# Autodesk Inventor assembly: finalassy
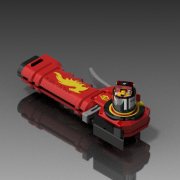
[picture p0: Inventor's stored thumbnail of the model, 180x180]
Saved by Autodesk Inventor 2018 (Build 220112000, 112)
## iProperties
Created: 2019-02-22
Part Number: finalassy
Material: 一般
Document SubType Name: Assembly
Designer: ku_sk
Author: ku_sk
## Documents named in this file (21)
- E:\windows\Documents\Inventor\Content Center Files\bay shooter\parts\finalassy.iam
- E:\windows\Documents\Inventor\Content Center Files\bay shooter\parts\undercover_modified.ipt
- E:\windows\Documents\Inventor\Content Center Files\bay shooter\parts\battery.ipt
- E:\windows\Documents\Inventor\Content Center Files\bay shooter\parts\brake.ipt
- E:\windows\Documents\Inventor\Content Center Files\bay shooter\parts\bay conect.ipt
- E:\windows\Documents\Inventor\Content Center Files\bay shooter\parts\bearing.ipt
- E:\windows\Documents\Inventor\Content Center Files\bay shooter\parts\bar.ipt
- E:\windows\Documents\Inventor\Content Center Files\bay shooter\parts\topcover.ipt
- E:\windows\Documents\Inventor\Content Center Files\bay shooter\parts\bar2.ipt
- E:\windows\Documents\Inventor\Content Center Files\bay shooter\parts\joint.ipt
- E:\windows\Documents\Inventor\Content Center Files\bay shooter\parts\switch.ipt
- E:\windows\Documents\Inventor\Content Center Files\bay shooter\parts\cover.ipt
- E:\windows\Documents\Inventor\Content Center Files\bay shooter\parts\ring.ipt
- E:\windows\Documents\Inventor\Content Center Files\bay shooter\parts\circuitcover.ipt
- E:\windows\Documents\Inventor\Content Center Files\bay shooter\parts\circuitcover1.ipt
- E:\windows\Documents\Inventor\Content Center Files\bay shooter\parts\gear.ipt
- E:\windows\Documents\Inventor\Content Center Files\bay shooter\parts\dragon.ipt
- E:\windows\Documents\Inventor\Content Center Files\bay shooter\parts\dragon_MIR.ipt
- E:\windows\Documents\Inventor\Content Center Files\bay shooter\parts\skyrimlogo2_1_9.ipt
- E:\windows\Documents\Inventor\Content Center Files\bay shooter\parts\pushbar.ipt
- E:\windows\Documents\Inventor\Content Center Files\bay shooter\reedy_540_rc_motor-1.snapshot.2\motor.iam
## Components (23 placed, 20 different names)
1. undercover_modified:1 — メイト:1, メイト:2, メイト:3, メイト:4, メイト:5, メイト:6, メイト:7, フラッシュ:1, メイト:11, メイト:12, メイト:13, メイト:14, メイト:15, メイト:16, 正接:1, メイト:18, メイト:22, メイト:27, メイト:33, メイト:34, メイト:35, メイト:43, メイト:44, メイト:45, メイト:46, メイト:47, メイト:48
2. battery:1 — メイト:4, メイト:5, メイト:6
3. bay conect:1 — メイト:7, メイト:8, メイト:9, メイト:10, メイト:19, フラッシュ:2
4. gear:1 — メイト:40, フラッシュ:2
5. bearing:1 — メイト:8, メイト:9, フラッシュ:1, メイト:20
6. bar:1 — メイト:10, メイト:16, メイト:17, メイト:21, メイト:23, メイト:26
7. topcover:1 — メイト:11, メイト:12, メイト:13, メイト:14, メイト:15, メイト:22, メイト:28, メイト:29, メイト:30, メイト:31, メイト:32, メイト:40, メイト:49, 角度:1, メイト:50, メイト:53, メイト:54, メイト:55
8. bar2:1 — メイト:19, メイト:20, メイト:21
9. joint:1 — メイト:23, メイト:24, メイト:25, メイト:26
10. switch:1 — メイト:24, メイト:25, メイト:27, メイト:51, フラッシュ:4, メイト:52
11. cover:1 — メイト:30, メイト:31, メイト:32
12. ring:1 — メイト:28, メイト:29
13. circuitcover:1 — メイト:33, メイト:34, メイト:35, メイト:36, メイト:37, メイト:38, メイト:39
14. circuitcover1:1 — メイト:36, メイト:37, メイト:38, メイト:39
15. dragon:1 — メイト:43, メイト:44, メイト:45
16. dragon_MIR:1 — メイト:46, メイト:47, メイト:48
17. skyrimlogo2_1_9:1 — メイト:49, 角度:1, メイト:50
18. pushbar:1 — メイト:51, フラッシュ:4, メイト:52
19. motor:1 [sub-assembly] — メイト:53, メイト:54, メイト:55
20. brake:1 — メイト:17, 正接:1, メイト:18
21. brake:2
22. brake:3
23. brake:4
## Component patterns: (4 elements, first: brake:1)
## Relationships (58: Mate 53, Flush 3, Tangent 1, Angle 1)
- メイト:1 [Mate]: undercover_modified:1
- メイト:2 [Mate]: undercover_modified:1
- メイト:3 [Mate]: undercover_modified:1
- メイト:4 [Mate] (0.5 mm): undercover_modified:1 ↔ battery:1
- メイト:5 [Mate] (0.5 mm): undercover_modified:1 ↔ battery:1
- メイト:6 [Mate]: undercover_modified:1 ↔ battery:1
- メイト:7 [Mate]: undercover_modified:1 ↔ bay conect:1
- メイト:8 [Mate]: bay conect:1 ↔ bearing:1
- メイト:9 [Mate]: bay conect:1 ↔ bearing:1
- フラッシュ:1 [Flush]: undercover_modified:1 ↔ bearing:1
- メイト:10 [Mate]: bay conect:1 ↔ bar:1
- メイト:11 [Mate]: undercover_modified:1 ↔ topcover:1
- メイト:12 [Mate]: undercover_modified:1 ↔ topcover:1
- メイト:13 [Mate]: undercover_modified:1 ↔ topcover:1
- メイト:14 [Mate]: undercover_modified:1 ↔ topcover:1
- メイト:15 [Mate]: undercover_modified:1 ↔ topcover:1
- メイト:16 [Mate]: undercover_modified:1 ↔ bar:1
- メイト:17 [Mate]: bar:1 ↔ brake:1
- 正接:1 [Tangent]: undercover_modified:1 ↔ brake:1
- メイト:18 [Mate]: undercover_modified:1 ↔ brake:1
- メイト:19 [Mate]: bay conect:1 ↔ bar2:1
- メイト:20 [Mate]: bearing:1 ↔ bar2:1
- メイト:21 [Mate]: bar:1 ↔ bar2:1
- メイト:22 [Mate]: undercover_modified:1 ↔ topcover:1
- メイト:23 [Mate]: bar:1 ↔ joint:1
- メイト:24 [Mate]: joint:1 ↔ switch:1
- メイト:25 [Mate] (0.25 mm): joint:1 ↔ switch:1
- メイト:26 [Mate]: bar:1 ↔ joint:1
- メイト:27 [Mate] (0.5 mm): undercover_modified:1 ↔ switch:1
- メイト:28 [Mate]: topcover:1 ↔ ring:1
- メイト:29 [Mate]: topcover:1 ↔ ring:1
- メイト:30 [Mate]: topcover:1 ↔ cover:1
- メイト:31 [Mate]: topcover:1 ↔ cover:1
- メイト:32 [Mate]: topcover:1 ↔ cover:1
- メイト:33 [Mate]: undercover_modified:1 ↔ circuitcover:1
- メイト:34 [Mate]: undercover_modified:1 ↔ circuitcover:1
- メイト:35 [Mate]: undercover_modified:1 ↔ circuitcover:1
- メイト:36 [Mate]: circuitcover:1 ↔ circuitcover1:1
- メイト:37 [Mate]: circuitcover:1 ↔ circuitcover1:1
- メイト:38 [Mate]: circuitcover:1 ↔ circuitcover1:1
- メイト:39 [Mate]: circuitcover:1 ↔ circuitcover1:1
- メイト:40 [Mate]: gear:1 ↔ topcover:1
- フラッシュ:2 [Flush]: bay conect:1 ↔ gear:1
- メイト:43 [Mate]: undercover_modified:1 ↔ dragon:1
- メイト:44 [Mate]: undercover_modified:1 ↔ dragon:1
- メイト:45 [Mate]: undercover_modified:1 ↔ dragon:1
- メイト:46 [Mate]: undercover_modified:1 ↔ dragon_MIR:1
- メイト:47 [Mate]: undercover_modified:1 ↔ dragon_MIR:1
- メイト:48 [Mate]: undercover_modified:1 ↔ dragon_MIR:1
- メイト:49 [Mate]: topcover:1 ↔ skyrimlogo2_1_9:1
- 角度:1 [Angle] (26.37 deg): topcover:1 ↔ skyrimlogo2_1_9:1
- メイト:50 [Mate]: topcover:1 ↔ skyrimlogo2_1_9:1
- メイト:51 [Mate]: switch:1 ↔ pushbar:1
- フラッシュ:4 [Flush]: switch:1 ↔ pushbar:1
- メイト:52 [Mate]: switch:1 ↔ pushbar:1
- メイト:53 [Mate]: topcover:1 ↔ motor:1
- メイト:54 [Mate]: topcover:1 ↔ motor:1
- メイト:55 [Mate]: topcover:1 ↔ motor:1
